# Autodesk Inventor assembly: RightNEX
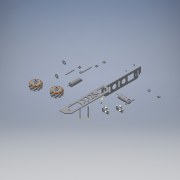
[picture p0: Inventor's stored thumbnail of the model, 180x180]
Saved by Autodesk Inventor 2017 (Build 210142000, 142)
## iProperties
Created: 2017-08-12
Part Number: RightNEX
Document SubType Name: Assembly
Designer: User
Author: User
## Documents named in this file (13)
- C:\Robotics\CAD\2016-17_CAD\DriveTrain\RightNEX.iam
- C:\Robotics\CAD\2016-17_CAD\DriveTrain\DriveTrainPlate2.0RightInside.ipt
- C:\Robotics\CAD\2016-17_CAD\DriveTrain\DriveTrainPlate2.0RightOutside.iam
- C:\Robotics\CAD\2016-17_CAD\DriveTrain\drive train standoff.ipt
- C:\Robotics\CAD\COTSParts\Motors\Andymark 2964  NeveRest 40 Motor.ipt
- C:\Robotics\CAD\COTSParts\Wheels\AndyMark Mecanum Wheels\100mm Aluminum Mecanum wheels.ipt
- C:\Robotics\CAD\COTSParts\Actobotics\545 parts\545556.ipt
- C:\Robotics\CAD\COTSParts\Actobotics\545 parts\545456.ipt
- C:\Robotics\CAD\COTSParts\Actobotics\535 parts\535198.ipt
- C:\Robotics\CAD\COTSParts\Actobotics\615 parts\615102.ipt
- C:\Robotics\CAD\COTSParts\Actobotics\634 parts\634080.ipt
- C:\Robotics\CAD\COTSParts\Tetrix\tetrix-motor-mounts-1.snapshot.1\Tetrex 2pc motor mount.ipt
- C:\Robotics\CAD\COTSParts\Actobotics\collar.ipt
## Components (35 placed, 12 different names)
1. DriveTrainPlate2.0RightInside:1
2. DriveTrainPlate2.0RightOutside:1 [sub-assembly]
3. drive train standoff:1
4. drive train standoff:2
5. drive train standoff:3
6. Andymark 2964  NeveRest 40 Motor:1
7. Andymark 2964  NeveRest 40 Motor:2
8. 100mm Aluminum Mecanum wheels:1 — Mate:7
9. 100mm Aluminum Mecanum wheels:2 — Mate:3, Mate:4
10. 545556:1
11. 545556:2 — Insert:1, Mate:6
12. 545556:3 — Insert:3, Mate:10
13. 545556:4
14. 545456:1
15. 545456:2 — Mate:3, Mate:4, Mate:5, Insert:1
16. 545456:3
17. 545456:4 — Mate:7, Mate:8, Mate:9
18. 535198:1
19. 535198:2
20. 535198:3 — Insert:2
21. 535198:4 — Mate:11
22. 615102:1
23. 615102:2 — Mate:5
24. 615102:3 — Mate:8, Mate:9, Insert:3
25. 615102:4
26. 545556:5
27. 545556:6
28. 634080:1
29. 634080:2
30. Tetrex 2pc motor mount:1
31. Tetrex 2pc motor mount:2
32. collar:1 — Mate:6, Insert:2
33. collar:2
34. collar:3
35. collar:4 — Mate:10, Mate:11
## Relationships (12: Mate 9, Insert 3)
- Mate:3: 100mm Aluminum Mecanum wheels:2 ↔ 545456:2
- Mate:4: 100mm Aluminum Mecanum wheels:2 ↔ 545456:2
- Mate:5: 545456:2 ↔ 615102:2
- Insert:1: 545556:2 ↔ 545456:2
- Mate:6: 545556:2 ↔ collar:1
- Insert:2: 535198:3 ↔ collar:1
- Mate:7: 100mm Aluminum Mecanum wheels:1 ↔ 545456:4
- Mate:8: 545456:4 ↔ 615102:3
- Mate:9: 545456:4 ↔ 615102:3
- Insert:3: 545556:3 ↔ 615102:3
- Mate:10: 545556:3 ↔ collar:4
- Mate:11: 535198:4 ↔ collar:4
